# Autodesk Inventor assembly: Vince-Motor
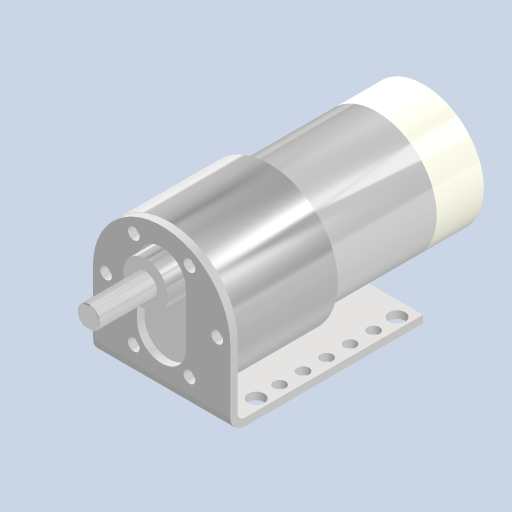
[picture p0: Inventor's stored thumbnail of the model, 512x512]
Saved by Autodesk Inventor 2024 (Build 280153000, 153)
## iProperties
Created: 2023-12-18
Part Number: Vince-Motor
Document SubType Name: Assembly
Designer: greg
Author: greg
## Documents named in this file (3)
- C:\Users\Greg\Documents\Inventor\Capstone\Chalk Applicator\Vince-Motor.iam
- C:\Users\Greg\Documents\Inventor\Capstone\Chalk Applicator\Vince-Motor.ipt
- C:\Users\Greg\Documents\Inventor\Capstone\Chalk Applicator\Vince-Motor-Bracket.ipt
## Components (2 placed, 2 different names)
1. Vince-Motor:1 — Mate:1, Mate:2, Insert:1
2. Vince-Motor-Bracket:1 — Mate:1, Mate:2, Insert:1
## Relationships (3: Mate 2, Insert 1)
- Mate:1: Vince-Motor:1 ↔ Vince-Motor-Bracket:1
- Mate:2: Vince-Motor:1 ↔ Vince-Motor-Bracket:1
- Insert:1: Vince-Motor:1 ↔ Vince-Motor-Bracket:1
